# Autodesk Inventor assembly: ROBOT
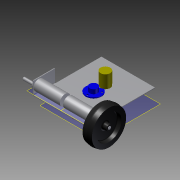
[picture p0: Inventor's stored thumbnail of the model, 180x180]
Saved by Autodesk Inventor 2014 (Build 180170000, 170)
## iProperties
Created: 2014-02-18
Part Number: ROBOT
Document SubType Name: Assembly
Designer: Pinkponk
Author: Pinkponk
## Documents named in this file (3)
- X:\Projekt\Min Robot\Min Robot\ROBOT.iam
- X:\Projekt\Min Robot\Min Robot\Motor Modul.iam
- X:\Projekt\Min Robot\Min Robot\Sensor Modul.iam
## Components (2 placed, 2 different names)
1. Motor Modul:1 [sub-assembly] — Insert:1, Insert:2
2. Sensor Modul:1 [sub-assembly] — Insert:1, Insert:2, Flush:1
## Relationships (3: Insert 2, Flush 1)
- Insert:1: Motor Modul:1 ↔ Sensor Modul:1
- Insert:2: Motor Modul:1 ↔ Sensor Modul:1
- Flush:1 (38.25 mm): Sensor Modul:1
